# Autodesk Inventor assembly: RC Assembly
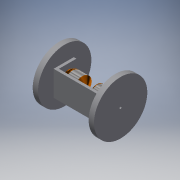
[picture p0: Inventor's stored thumbnail of the model, 180x180]
Saved by Autodesk Inventor 2019.2 (Build 232265000, 265)
## iProperties
Created: 2019-05-20
Part Number: RC Assembly
Document SubType Name: Assembly
Designer: Johansson
Author: Johansson
## Documents named in this file (4)
- D:\Dropbox\Dokument\Projekt\RC Two Wheeler\RC-two-wheeler\CAD\RC Assembly.iam
- D:\Dropbox\Dokument\Projekt\RC Two Wheeler\RC-two-wheeler\CAD\KEDA_6364.ipt
- D:\Dropbox\Dokument\Projekt\RC Two Wheeler\RC-two-wheeler\CAD\Platform.ipt
- D:\Dropbox\Dokument\Projekt\RC Two Wheeler\RC-two-wheeler\CAD\Wheel.ipt
## Components (5 placed, 3 different names)
1. KEDA_6364:1 — Mate:1, Mate:2, Mate:3, Cylindrical:2, Mate:7
2. Platform:1 — Mate:1, Mate:2, Mate:3, Mate:4, Mate:5, Mate:6
3. KEDA_6364:2 — Mate:4, Mate:5, Mate:6, Cylindrical:1, Mate:8
4. Wheel:1 — Cylindrical:2, Mate:7
5. Wheel:2 — Cylindrical:1, Mate:8
## Relationships (10: Mate 8, CylindricalJoint 2)
- Mate:1: KEDA_6364:1 ↔ Platform:1
- Mate:2: KEDA_6364:1 ↔ Platform:1
- Mate:3: KEDA_6364:1 ↔ Platform:1
- Mate:4: Platform:1 ↔ KEDA_6364:2
- Mate:5: Platform:1 ↔ KEDA_6364:2
- Mate:6: Platform:1 ↔ KEDA_6364:2
- Cylindrical:1: KEDA_6364:2 ↔ Wheel:2
- Cylindrical:2: KEDA_6364:1 ↔ Wheel:1
- Mate:7 (-10 mm): KEDA_6364:1 ↔ Wheel:1
- Mate:8 (-10 mm): KEDA_6364:2 ↔ Wheel:2
